# Autodesk Inventor assembly: ASY MSC 080 gills
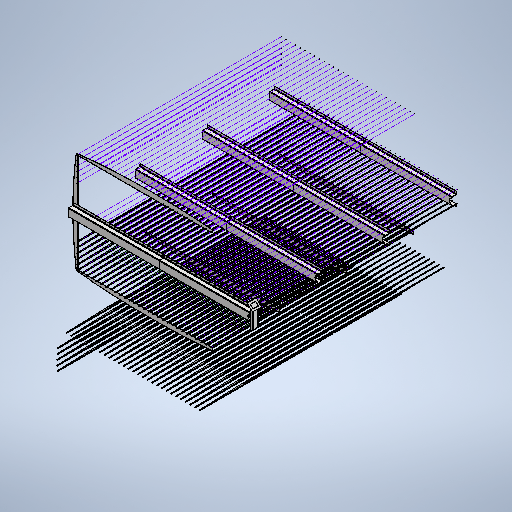
[picture p0: Inventor's stored thumbnail of the model, 512x512]
Saved by Autodesk Inventor 2025 (Build 290162010, 162A)
## iProperties
Created: 2024-08-31
Part Number: ASY MSC 080 gills
Document SubType Name: Assembly
Designer: pokla
Stock Number: ASY МОО 080 Жабры
Author: pokla
## Documents named in this file (19)
- C:\Users\user\YandexDisk\домашниий пк\Inventor\Manturovo\Manturovo_Se-clar\ASY MSC 080 gills.iam
- C:\Users\user\YandexDisk\домашниий пк\Inventor\Manturovo\Manturovo_Se-clar\MSC 802 sheet gills.ipt
- C:\Users\user\YandexDisk\домашниий пк\Inventor\Manturovo\Manturovo_Se-clar\MSC 081 pillar gills.ipt
- C:\Users\user\YandexDisk\домашниий пк\Inventor\Manturovo\Manturovo_Se-clar\MSC 804 sheet gills.ipt
- C:\Users\user\YandexDisk\домашниий пк\Inventor\Manturovo\Manturovo_Se-clar\MSC 803 sheet gills.ipt
- C:\Users\user\YandexDisk\домашниий пк\Inventor\Manturovo\Manturovo_Se-clar\MSC 806 sheet gills.ipt
- C:\Users\user\YandexDisk\домашниий пк\Inventor\Manturovo\Manturovo_Se-clar\MSC 805 sheet gills.ipt
- C:\Users\user\YandexDisk\домашниий пк\Inventor\Manturovo\Manturovo_Se-clar\MSC 808 sheet gills.ipt
- C:\Users\user\YandexDisk\домашниий пк\Inventor\Manturovo\Manturovo_Se-clar\MSC 807 sheet gills.ipt
- C:\Users\user\YandexDisk\домашниий пк\Inventor\Manturovo\Manturovo_Se-clar\MSC 810 sheet gills.ipt
- C:\Users\user\YandexDisk\домашниий пк\Inventor\Manturovo\Manturovo_Se-clar\MSC 809 sheet gills.ipt
- C:\Users\user\YandexDisk\домашниий пк\Inventor\Manturovo\Manturovo_Se-clar\MSC 812 sheet gills.ipt
- C:\Users\user\YandexDisk\домашниий пк\Inventor\Manturovo\Manturovo_Se-clar\MSC 811 sheet gills.ipt
- C:\Users\user\YandexDisk\домашниий пк\Inventor\Manturovo\Manturovo_Se-clar\MSC 084 wall support gills.ipt
- C:\Users\user\YandexDisk\домашниий пк\Inventor\Manturovo\Manturovo_Se-clar\MSC 082 pillar gills.ipt
- C:\Users\user\YandexDisk\домашниий пк\Inventor\Manturovo\Manturovo_Se-clar\MSC 086 string for sheets gills.ipt
- C:\Users\user\YandexDisk\домашниий пк\Inventor\Manturovo\Manturovo_Se-clar\MSC 083 top support gills.ipt
- C:\Users\user\YandexDisk\домашниий пк\Inventor\Manturovo\Manturovo_Se-clar\MSC 801 sheet gills.ipt
- C:\Users\user\YandexDisk\домашниий пк\Inventor\Manturovo\Manturovo_Se-clar\ASY MSC 089 gills base.iam
## Components (288 placed, 29 different names)
1. MSC 804 sheet gills:1 — Rigid:39
2. MSC 803 sheet gills:1 — Angle:2, Tangent:8, Tangent:9, Flush:15, Flush:19, Rigid:39
3. MSC 806 sheet gills:1 — Rigid:36
4. MSC 805 sheet gills:1 — Rigid:36, Angle:3, Tangent:10, Tangent:11, Flush:15, Flush:16
5. MSC 808 sheet gills:1 — Rigid:37
6. MSC 807 sheet gills:1 — Rigid:37, Angle:4, Tangent:12, Tangent:13, Flush:16, Flush:17
7. MSC 810 sheet gills:1 — Rigid:38
8. MSC 809 sheet gills:1 — Rigid:38, Angle:5, Tangent:17, Tangent:18, Flush:17, Flush:18
9. MSC 812 sheet gills:1 — Rigid:32
10. MSC 811 sheet gills:1 — Rigid:32, Angle:6, Tangent:19, Tangent:20, Flush:18
11. MSC 084 wall support gills:1 — Rigid:12, Rigid:25, Rigid:30, Tangent:14, Tangent:15
12. MSC 084 wall support gills:2 — Rigid:25, Rigid:26, Mate:17
13. MSC 084 wall support gills:3 — Rigid:26, Rigid:27
14. MSC 084 wall support gills:4 — Rigid:27
15. MSC 083 top support gills:2 — Rigid:28, Rigid:30, Tangent:8, Tangent:9, Tangent:10, Tangent:11, Tangent:12, Tangent:13, Tangent:17, Tangent:18, Tangent:19, Tangent:20, Rigid:40
16. MSC 083 top support gills:1 — Rigid:24, Rigid:29, Rigid:31
17. MSC 084 wall support gills:5 — Rigid:15, Rigid:31
18. MSC 0103 sheet gills:2
19. MSC 0203 sheet gills:2
20. MSC 0104 sheet gills:2
21. MSC 0204 sheet gills:2
22. MSC 0105 sheet gills:2
23. MSC 0205 sheet gills:2
24. MSC 0106 sheet gills:2
25. MSC 0206 sheet gills:2
26. MSC 0107 sheet gills:2
27. MSC 0207 sheet gills:2
28. ASY MSC 089 gills base:1 [sub-assembly]
29. MSC 081 pillar gills:1 — Rotational:1, Rotational:2, Tangent:16
30. MSC 082 pillar gills:1 — Rigid:28, Rigid:29
31. MSC 081 pillar gills:2
32. MSC 082 pillar gills:2
33. MSC 081 pillar gills:3
34. MSC 082 pillar gills:3
35. MSC 081 pillar gills:4
36. MSC 082 pillar gills:4
37. MSC 801 sheet gills:1 — Mate:17, Rigid:33, Angle:2, Angle:3, Angle:4, Angle:5, Angle:6, Tangent:14, Tangent:15, Tangent:16, Flush:19
38. MSC 802 sheet gills:1 — Rigid:33
39. MSC 802 sheet gills:2
40. MSC 0201 sheet gills:2
41. MSC 0201 sheet gills:3
42. MSC 802 sheet gills:3
43. MSC 802 sheet gills:4
44. MSC 0201 sheet gills:4
45. MSC 0201 sheet gills:5
46. MSC 802 sheet gills:5
47. MSC 802 sheet gills:6
48. MSC 0201 sheet gills:6
49. MSC 0201 sheet gills:7
50. MSC 802 sheet gills:7
51. MSC 802 sheet gills:8
52. MSC 0201 sheet gills:8
53. MSC 0201 sheet gills:9
54. MSC 802 sheet gills:9
55. MSC 802 sheet gills:10
56. MSC 0201 sheet gills:10
57. MSC 0201 sheet gills:11
58. MSC 802 sheet gills:11
59. MSC 802 sheet gills:12
60. MSC 0201 sheet gills:12
61. MSC 0201 sheet gills:13
62. MSC 802 sheet gills:13
63. MSC 802 sheet gills:14
64. MSC 0201 sheet gills:14
65. MSC 0201 sheet gills:15
66. MSC 802 sheet gills:15
67. MSC 802 sheet gills:16
68. MSC 0201 sheet gills:16
69. MSC 0201 sheet gills:17
70. MSC 802 sheet gills:17
71. MSC 802 sheet gills:18
72. MSC 0201 sheet gills:18
73. MSC 0201 sheet gills:19
74. MSC 802 sheet gills:19
75. MSC 802 sheet gills:20
76. MSC 0201 sheet gills:20
77. MSC 0201 sheet gills:21
78. MSC 802 sheet gills:21
79. MSC 802 sheet gills:22
80. MSC 0201 sheet gills:22
81. MSC 0201 sheet gills:23
82. MSC 802 sheet gills:23
83. MSC 802 sheet gills:24
84. MSC 0201 sheet gills:24
85. MSC 0201 sheet gills:25
86. MSC 802 sheet gills:25
87. MSC 802 sheet gills:26
88. MSC 0201 sheet gills:26
89. MSC 0201 sheet gills:27
90. MSC 802 sheet gills:27
91. MSC 802 sheet gills:28
92. MSC 0201 sheet gills:28
93. MSC 0201 sheet gills:29
94. MSC 802 sheet gills:29
95. MSC 802 sheet gills:30
96. MSC 0201 sheet gills:30
97. MSC 0201 sheet gills:31
98. MSC 802 sheet gills:31
99. MSC 802 sheet gills:32
100. MSC 0201 sheet gills:32
101. MSC 0201 sheet gills:33
102. MSC 802 sheet gills:33
103. MSC 802 sheet gills:34
104. MSC 0201 sheet gills:34
105. MSC 0201 sheet gills:35
106. MSC 802 sheet gills:35
107. MSC 802 sheet gills:36
108. MSC 0201 sheet gills:36
109. MSC 0201 sheet gills:37
110. MSC 802 sheet gills:37
111. MSC 802 sheet gills:38
112. MSC 0201 sheet gills:38
113. MSC 0201 sheet gills:39
114. MSC 802 sheet gills:39
115. MSC 802 sheet gills:40
116. MSC 0201 sheet gills:40
117. MSC 0201 sheet gills:41
118. MSC 802 sheet gills:41
119. MSC 802 sheet gills:42
120. MSC 0201 sheet gills:42
121. MSC 0201 sheet gills:43
122. MSC 802 sheet gills:43
123. MSC 802 sheet gills:44
124. MSC 0201 sheet gills:44
125. MSC 0201 sheet gills:45
126. MSC 802 sheet gills:45
127. MSC 802 sheet gills:46
128. MSC 0201 sheet gills:46
129. MSC 0201 sheet gills:47
130. MSC 802 sheet gills:47
131. MSC 802 sheet gills:48
132. MSC 0201 sheet gills:48
133. MSC 0201 sheet gills:49
134. MSC 802 sheet gills:49
135. MSC 802 sheet gills:50
136. MSC 0201 sheet gills:50
137. MSC 0201 sheet gills:51
138. MSC 802 sheet gills:51
139. MSC 802 sheet gills:52
140. MSC 0201 sheet gills:52
141. MSC 0201 sheet gills:53
142. MSC 802 sheet gills:53
143. MSC 802 sheet gills:54
144. MSC 0201 sheet gills:54
145. MSC 0201 sheet gills:55
146. MSC 802 sheet gills:55
147. MSC 802 sheet gills:56
148. MSC 0201 sheet gills:56
149. MSC 0201 sheet gills:57
150. MSC 802 sheet gills:57
151. MSC 802 sheet gills:58
152. MSC 0201 sheet gills:58
153. MSC 086 string for sheets gills:1 — Rigid:12
154. MSC 086 string for sheets gills:2 — Rigid:15
155. MSC 086 string for sheets gills:3
156. MSC 086 string for sheets gills:344
157. MSC 086 string for sheets gills:5
158. MSC 086 string for sheets gills:345
159. MSC 086 string for sheets gills:7
160. MSC 086 string for sheets gills:346
161. MSC 086 string for sheets gills:9
162. MSC 086 string for sheets gills:347
163. MSC 086 string for sheets gills:11
164. MSC 086 string for sheets gills:348
165. MSC 086 string for sheets gills:13
166. MSC 086 string for sheets gills:349
167. MSC 086 string for sheets gills:15
168. MSC 086 string for sheets gills:350
169. MSC 086 string for sheets gills:17
170. MSC 086 string for sheets gills:351
171. MSC 086 string for sheets gills:19
172. MSC 086 string for sheets gills:352
173. MSC 086 string for sheets gills:21
174. MSC 086 string for sheets gills:353
175. MSC 086 string for sheets gills:23
176. MSC 086 string for sheets gills:354
177. MSC 086 string for sheets gills:25
178. MSC 086 string for sheets gills:355
179. MSC 086 string for sheets gills:27
180. MSC 086 string for sheets gills:356
181. MSC 086 string for sheets gills:29
182. MSC 086 string for sheets gills:357
183. MSC 086 string for sheets gills:31
184. MSC 086 string for sheets gills:358
185. MSC 086 string for sheets gills:33
186. MSC 086 string for sheets gills:359
187. MSC 086 string for sheets gills:35
188. MSC 086 string for sheets gills:360
189. MSC 086 string for sheets gills:37
190. MSC 086 string for sheets gills:361
191. MSC 086 string for sheets gills:39
192. MSC 086 string for sheets gills:362
193. MSC 086 string for sheets gills:41
194. MSC 086 string for sheets gills:363
195. MSC 086 string for sheets gills:43
196. MSC 086 string for sheets gills:364
197. MSC 086 string for sheets gills:45
198. MSC 086 string for sheets gills:365
199. MSC 086 string for sheets gills:47
200. MSC 086 string for sheets gills:366
201. MSC 086 string for sheets gills:49
202. MSC 086 string for sheets gills:367
203. MSC 086 string for sheets gills:51
204. MSC 086 string for sheets gills:368
205. MSC 086 string for sheets gills:53
206. MSC 086 string for sheets gills:369
207. MSC 086 string for sheets gills:55
208. MSC 086 string for sheets gills:370
209. MSC 086 string for sheets gills:58 — Rotational:1
210. MSC 086 string for sheets gills:57 — Rotational:2
211. MSC 086 string for sheets gills:278
212. MSC 086 string for sheets gills:279
213. MSC 086 string for sheets gills:280
214. MSC 086 string for sheets gills:281
215. MSC 086 string for sheets gills:282
216. MSC 086 string for sheets gills:283
217. MSC 086 string for sheets gills:284
218. MSC 086 string for sheets gills:285
219. MSC 086 string for sheets gills:286
220. MSC 086 string for sheets gills:287
221. MSC 086 string for sheets gills:288
222. MSC 086 string for sheets gills:289
223. MSC 086 string for sheets gills:290
224. MSC 086 string for sheets gills:291
225. MSC 086 string for sheets gills:292
226. MSC 086 string for sheets gills:293
227. MSC 086 string for sheets gills:294
228. MSC 086 string for sheets gills:295
229. MSC 086 string for sheets gills:296
230. MSC 086 string for sheets gills:297
231. MSC 086 string for sheets gills:298
232. MSC 086 string for sheets gills:299
233. MSC 086 string for sheets gills:300
234. MSC 086 string for sheets gills:301
235. MSC 086 string for sheets gills:302
236. MSC 086 string for sheets gills:303
237. MSC 086 string for sheets gills:304
238. MSC 086 string for sheets gills:305
239. MSC 086 string for sheets gills:306
240. MSC 086 string for sheets gills:307
241. MSC 086 string for sheets gills:308
242. MSC 086 string for sheets gills:309
243. MSC 086 string for sheets gills:310
244. MSC 086 string for sheets gills:311
245. MSC 086 string for sheets gills:312
246. MSC 086 string for sheets gills:313
247. MSC 086 string for sheets gills:314
248. MSC 086 string for sheets gills:315
249. MSC 086 string for sheets gills:316
250. MSC 086 string for sheets gills:317
251. MSC 086 string for sheets gills:318
252. MSC 086 string for sheets gills:319
253. MSC 086 string for sheets gills:320
254. MSC 086 string for sheets gills:321
255. MSC 086 string for sheets gills:322
256. MSC 086 string for sheets gills:323
257. MSC 086 string for sheets gills:324
258. MSC 086 string for sheets gills:325
259. MSC 086 string for sheets gills:326
260. MSC 086 string for sheets gills:327
261. MSC 086 string for sheets gills:328
262. MSC 086 string for sheets gills:329
263. MSC 086 string for sheets gills:330
264. MSC 086 string for sheets gills:331
265. MSC 086 string for sheets gills:332
266. MSC 086 string for sheets gills:333
267. MSC 086 string for sheets gills:334
268. MSC 086 string for sheets gills:335
269. MSC 086 string for sheets gills:336
270. MSC 086 string for sheets gills:337
271. MSC 086 string for sheets gills:338
272. MSC 086 string for sheets gills:339
273. MSC 086 string for sheets gills:340
274. MSC 086 string for sheets gills:341
275. MSC 086 string for sheets gills:342
276. MSC 086 string for sheets gills:343
277. MSC 086 string for sheets gills:125 — Rigid:40
278. MSC 086 string for sheets gills:126
279. MSC 086 string for sheets gills:127
280. MSC 086 string for sheets gills:128
281. MSC 086 string for sheets gills:129
282. MSC 086 string for sheets gills:130
283. MSC 086 string for sheets gills:131 — Rigid:24
284. MSC 086 string for sheets gills:371
285. MSC 086 string for sheets gills:372
286. MSC 086 string for sheets gills:373
287. MSC 086 string for sheets gills:374
288. MSC 086 string for sheets gills:375
## Component patterns: (4 elements, first: MSC 081 pillar gills:1 + MSC 082 pillar gills:1), (29 elements, first: MSC 801 sheet gills:1 + MSC 802 sheet gills:1 + MSC 802 sheet gills:2 + MSC 0201 sheet gills:2), (28 elements, first: MSC 086 string for sheets gills:1 + MSC 086 string for sheets gills:2), (34 elements, first: MSC 086 string for sheets gills:58 + MSC 086 string for sheets gills:57), (6 elements, first: MSC 086 string for sheets gills:125), (6 elements, first: MSC 086 string for sheets gills:131)
## Relationships (60: WeldJoint 24, Tangent 13, Flush 12, Angle 5, Mate 4, RevoluteJoint 2)
- [WeldJoint]: MSC 081 pillar gills:1 ↔ MSC 082 pillar gills:1
- [Flush]: ASY MSC 089 gills base:1 ↔ MSC 081 pillar gills:1
- [Mate]: ASY MSC 089 gills base:1 ↔ MSC 081 pillar gills:1
- [Flush] (5 mm): ASY MSC 089 gills base:1 ↔ MSC 081 pillar gills:1
- Rigid:12 [WeldJoint] (-5 mm): MSC 084 wall support gills:1 ↔ MSC 086 string for sheets gills:1
- Rigid:15 [WeldJoint] (-5 mm): MSC 084 wall support gills:5 ↔ MSC 086 string for sheets gills:2
- [Mate]: ASY MSC 089 gills base:1
- [Mate]: ASY MSC 089 gills base:1
- [Flush]: ASY MSC 089 gills base:1
- Rigid:24 [WeldJoint] (-5 mm): MSC 083 top support gills:1 ↔ MSC 086 string for sheets gills:131
- Rigid:25 [WeldJoint] (985 mm): MSC 084 wall support gills:1 ↔ MSC 084 wall support gills:2
- Rigid:26 [WeldJoint] (985 mm): MSC 084 wall support gills:2 ↔ MSC 084 wall support gills:3
- Rigid:27 [WeldJoint] (985 mm): MSC 084 wall support gills:3 ↔ MSC 084 wall support gills:4
- Mate:17: MSC 084 wall support gills:2 ↔ MSC 801 sheet gills:1
- Rigid:28 [WeldJoint]: MSC 083 top support gills:2 ↔ MSC 082 pillar gills:1
- Rigid:29 [WeldJoint]: MSC 083 top support gills:1 ↔ MSC 082 pillar gills:1
- Rigid:30 [WeldJoint]: MSC 084 wall support gills:1 ↔ MSC 083 top support gills:2
- Rigid:31 [WeldJoint]: MSC 083 top support gills:1 ↔ MSC 084 wall support gills:5
- Rotational:1 [RevoluteJoint] (5 mm): MSC 081 pillar gills:1 ↔ MSC 086 string for sheets gills:58
- Rotational:2 [RevoluteJoint] (-5 mm): MSC 081 pillar gills:1 ↔ MSC 086 string for sheets gills:57
- Rigid:32 [WeldJoint] (-10 mm): MSC 812 sheet gills:1 ↔ MSC 811 sheet gills:1
- Rigid:33 [WeldJoint] (-10 mm): MSC 801 sheet gills:1 ↔ MSC 802 sheet gills:1
- Rigid:36 [WeldJoint] (-10 mm): MSC 806 sheet gills:1 ↔ MSC 805 sheet gills:1
- Rigid:37 [WeldJoint] (-10 mm): MSC 808 sheet gills:1 ↔ MSC 807 sheet gills:1
- Rigid:38 [WeldJoint] (-10 mm): MSC 810 sheet gills:1 ↔ MSC 809 sheet gills:1
- Angle:2 (0 deg): MSC 803 sheet gills:1 ↔ MSC 801 sheet gills:1
- Angle:3 (0 deg): MSC 805 sheet gills:1 ↔ MSC 801 sheet gills:1
- Angle:4 (0 deg): MSC 807 sheet gills:1 ↔ MSC 801 sheet gills:1
- Angle:5 (0 deg): MSC 809 sheet gills:1 ↔ MSC 801 sheet gills:1
- Angle:6 (0 deg): MSC 811 sheet gills:1 ↔ MSC 801 sheet gills:1
- Tangent:8: MSC 803 sheet gills:1 ↔ MSC 083 top support gills:2
- Tangent:9: MSC 803 sheet gills:1 ↔ MSC 083 top support gills:2
- Tangent:10: MSC 805 sheet gills:1 ↔ MSC 083 top support gills:2
- Tangent:11: MSC 805 sheet gills:1 ↔ MSC 083 top support gills:2
- Tangent:12: MSC 807 sheet gills:1 ↔ MSC 083 top support gills:2
- Tangent:13: MSC 807 sheet gills:1 ↔ MSC 083 top support gills:2
- Tangent:14: MSC 084 wall support gills:1 ↔ MSC 801 sheet gills:1
- Tangent:15: MSC 084 wall support gills:1 ↔ MSC 801 sheet gills:1
- Tangent:16: MSC 081 pillar gills:1 ↔ MSC 801 sheet gills:1
- Tangent:17: MSC 809 sheet gills:1 ↔ MSC 083 top support gills:2
- Tangent:18: MSC 809 sheet gills:1 ↔ MSC 083 top support gills:2
- Tangent:19: MSC 811 sheet gills:1 ↔ MSC 083 top support gills:2
- Tangent:20: MSC 811 sheet gills:1 ↔ MSC 083 top support gills:2
- Flush:15: MSC 803 sheet gills:1 ↔ MSC 805 sheet gills:1
- Flush:16: MSC 805 sheet gills:1 ↔ MSC 807 sheet gills:1
- Flush:17: MSC 807 sheet gills:1 ↔ MSC 809 sheet gills:1
- Flush:18: MSC 809 sheet gills:1 ↔ MSC 811 sheet gills:1
- Flush:19: MSC 803 sheet gills:1 ↔ MSC 801 sheet gills:1
- Rigid:39 [WeldJoint] (-10 mm): MSC 804 sheet gills:1 ↔ MSC 803 sheet gills:1
- Rigid:40 [WeldJoint] (5 mm): MSC 083 top support gills:2 ↔ MSC 086 string for sheets gills:125
- [WeldJoint] (-10 mm): MSC 802 sheet gills:2 ↔ MSC 0201 sheet gills:2
- [WeldJoint] (-10 mm): MSC 0107 sheet gills:2 ↔ MSC 0207 sheet gills:2
- [WeldJoint] (-10 mm): MSC 0104 sheet gills:2 ↔ MSC 0204 sheet gills:2
- [WeldJoint] (-10 mm): MSC 0105 sheet gills:2 ↔ MSC 0205 sheet gills:2
- [WeldJoint] (-10 mm): MSC 0106 sheet gills:2 ↔ MSC 0206 sheet gills:2
- [Flush]: MSC 0203 sheet gills:2 ↔ MSC 0204 sheet gills:2
- [Flush]: MSC 0204 sheet gills:2 ↔ MSC 0205 sheet gills:2
- [Flush]: MSC 0205 sheet gills:2 ↔ MSC 0206 sheet gills:2
- [Flush]: MSC 0206 sheet gills:2 ↔ MSC 0207 sheet gills:2
- [WeldJoint] (-10 mm): MSC 0103 sheet gills:2 ↔ MSC 0203 sheet gills:2
## Named parameters: d233_d176 = -10 mm, d234_d202 = 0 mm, d235_d203 = 0 mm, d236_d204 = 0 mm, d237_d205 = 0 mm, d238_d207 = -10 mm, d239_d180 = -10 mm, d240_d181 = -10 mm, d241_d173 = -10 mm, d242_d179 = -10 mm
